# Autodesk Inventor assembly: ABCD Assemble
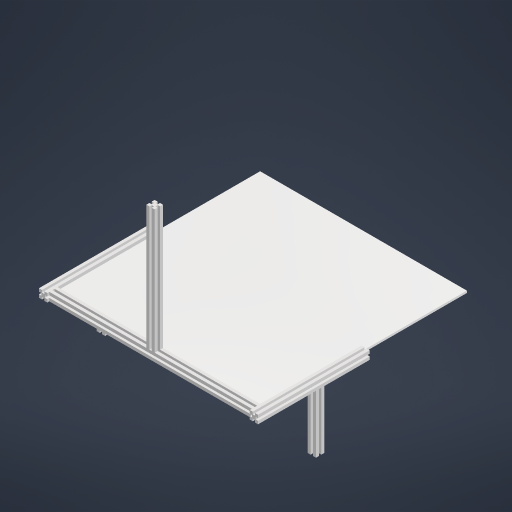
[picture p0: Inventor's stored thumbnail of the model, 512x512]
Saved by Autodesk Inventor 2024 (Build 280153000, 153)
## iProperties
Created: 2023-09-19
Part Number: ABCD Assemble
Document SubType Name: Assembly
Designer: 6gioc
Author: 6gioc
## Documents named in this file (3)
- C:\Users\6gioc\OneDrive\AAST\PART\ABCD\ABCD Assemble.iam
- C:\Users\6gioc\OneDrive\AAST\PART\ABCD\acrillboard.ipt
- C:\Users\6gioc\OneDrive\AAST\PART\ABCD\grabber.ipt
## Components (2 placed, 2 different names)
1. acrillboard:1 — 플러쉬:1
2. grabber:1 — 플러쉬:1
## Relationships (1: Flush 1)
- 플러쉬:1 [Flush]: acrillboard:1 ↔ grabber:1
